# Autodesk Inventor assembly: leftSide
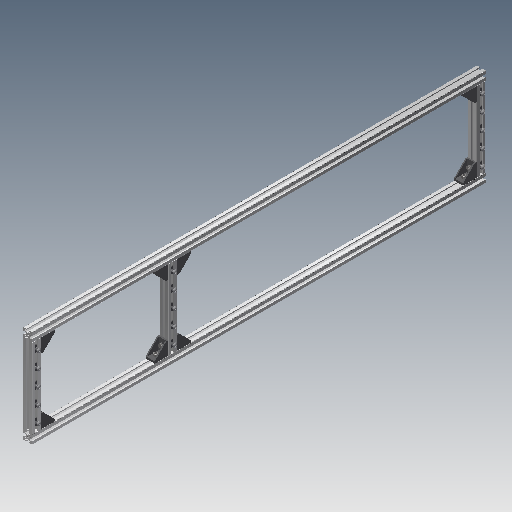
[picture p0: Inventor's stored thumbnail of the model, 512x512]
Saved by Autodesk Inventor 2017 (Build 210142000, 142)
## iProperties
Created: 2017-03-01
Part Number: leftSide
Document SubType Name: Assembly
Designer: sawaiz
Author: sawaiz
## Documents named in this file (5)
- C:\Users\sawaiz\oneDrive\projects\sPhenixTileTestStand\frame\leftSide.iam
- C:\Users\sawaiz\oneDrive\projects\sPhenixTileTestStand\frame\vertical.iam
- C:\Users\sawaiz\oneDrive\projects\sPhenixTileTestStand\frame\hfs5-2020Depth.ipt
- C:\Users\sawaiz\oneDrive\projects\sPhenixTileTestStand\hardware\angleBracket.iam
- C:\Users\sawaiz\oneDrive\projects\sPhenixTileTestStand\sPhenixTileTestStand.xlsx
## Components (13 placed, 3 different names)
1. vertical:1 [sub-assembly] — Flush:2, Flush:3, Flush:5, Flush:6, Mate:1, Mate:4, Flush:11, Mate:12
2. vertical:2 [sub-assembly] — Flush:1, Flush:2, Flush:3, Flush:4, Flush:8, Mate:13, Flush:21, Mate:14, Mate:17, Mate:18, Flush:26
3. vertical:3 [sub-assembly] — Flush:1, Flush:4, Flush:7, Flush:8, Flush:9, Flush:10, Mate:2, Mate:15, Mate:16
4. hfs5-2020Depth:1 — Flush:5, Flush:6, Mate:1, Flush:7, Symmetry:1, Symmetry:2, Symmetry:3, Mate:8, Mate:9, Mate:10, Flush:14, Mate:11
5. hfs5-2020Depth:2 — Flush:9, Flush:10, Mate:2, Symmetry:1, Symmetry:2, Symmetry:3, Mate:3, Flush:12, Mate:5, Mate:6, Mate:7
6. angleBracket:1 [sub-assembly] — Mate:7, Mate:15, Flush:25
7. angleBracket:2 [sub-assembly] — Mate:9, Flush:22, Mate:16
8. angleBracket:3 [sub-assembly] — Mate:6, Mate:14, Flush:22, Flush:23, Flush:25
9. angleBracket:4 [sub-assembly] — Mate:10, Mate:18, Flush:26, Flush:27
10. angleBracket:5 [sub-assembly] — Mate:5, Mate:13, Flush:21, Flush:23, Flush:24
11. angleBracket:6 [sub-assembly] — Mate:8, Flush:14, Mate:17, Flush:27
12. angleBracket:7 [sub-assembly] — Mate:4, Flush:11, Flush:20, Mate:11
13. angleBracket:8 [sub-assembly] — Mate:3, Flush:12, Flush:20, Mate:12, Flush:24
## Relationships (42: Flush 21, Mate 18, Symmetry 3)
- Flush:1: vertical:2 ↔ vertical:3
- Flush:2: vertical:1 ↔ vertical:2
- Flush:3: vertical:1 ↔ vertical:2
- Flush:4: vertical:2 ↔ vertical:3
- Flush:5: vertical:1 ↔ hfs5-2020Depth:1
- Flush:6: vertical:1 ↔ hfs5-2020Depth:1
- Mate:1: vertical:1 ↔ hfs5-2020Depth:1
- Flush:7: vertical:3 ↔ hfs5-2020Depth:1
- Flush:8 (300 mm): vertical:2 ↔ vertical:3
- Flush:9: vertical:3 ↔ hfs5-2020Depth:2
- Flush:10: vertical:3 ↔ hfs5-2020Depth:2
- Mate:2: vertical:3 ↔ hfs5-2020Depth:2
- Symmetry:1: hfs5-2020Depth:1 ↔ hfs5-2020Depth:2
- Symmetry:2: hfs5-2020Depth:1 ↔ hfs5-2020Depth:2
- Symmetry:3: hfs5-2020Depth:1 ↔ hfs5-2020Depth:2
- Mate:3: hfs5-2020Depth:2 ↔ angleBracket:8
- Mate:4: vertical:1 ↔ angleBracket:7
- Flush:11: vertical:1 ↔ angleBracket:7
- Flush:12: hfs5-2020Depth:2 ↔ angleBracket:8
- Mate:5: hfs5-2020Depth:2 ↔ angleBracket:5
- Mate:6: hfs5-2020Depth:2 ↔ angleBracket:3
- Mate:7: hfs5-2020Depth:2 ↔ angleBracket:1
- Mate:8: hfs5-2020Depth:1 ↔ angleBracket:6
- Mate:9: hfs5-2020Depth:1 ↔ angleBracket:2
- Mate:10: hfs5-2020Depth:1 ↔ angleBracket:4
- Flush:14: hfs5-2020Depth:1 ↔ angleBracket:6
- Flush:20: angleBracket:7 ↔ angleBracket:8
- Mate:11: hfs5-2020Depth:1 ↔ angleBracket:7
- Mate:12: vertical:1 ↔ angleBracket:8
- Mate:13: vertical:2 ↔ angleBracket:5
- Flush:21: vertical:2 ↔ angleBracket:5
- Mate:14: vertical:2 ↔ angleBracket:3
- Flush:22: angleBracket:2 ↔ angleBracket:3
- Flush:23: angleBracket:3 ↔ angleBracket:5
- Flush:24: angleBracket:5 ↔ angleBracket:8
- Mate:15: vertical:3 ↔ angleBracket:1
- Flush:25: angleBracket:1 ↔ angleBracket:3
- Mate:16: vertical:3 ↔ angleBracket:2
- Mate:17: vertical:2 ↔ angleBracket:6
- Mate:18: vertical:2 ↔ angleBracket:4
- Flush:26: vertical:2 ↔ angleBracket:4
- Flush:27: angleBracket:4 ↔ angleBracket:6
## Named parameters: plateWidth = 300 mm, plateDepth = 1000 mm, supportPlateThickness = 6.35 mm, supportPlateWidth = 50 mm, supportPlateFillet = 10 mm, separation = 35 mm, numPanels = 5, centerVerticalRatio = 0.3
